# Autodesk Inventor assembly: ASY MSC 080 roсket
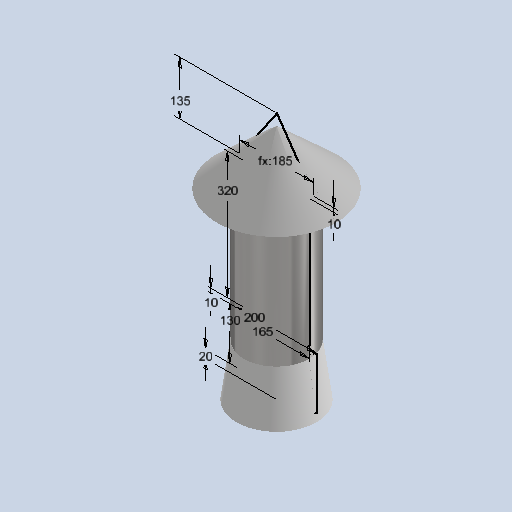
[picture p0: Inventor's stored thumbnail of the model, 512x512]
Saved by Autodesk Inventor 2024.2 (Build 282272000, 272)
## iProperties
Created: 2024-05-19
Part Number: ASY MSC 080 roсket
Document SubType Name: Assembly
Designer: admin
Stock Number: ASY МОО 080 ракета
Author: admin
## Documents named in this file (5)
- C:\Users\pokla\Documents\Inventor\Отстойник осветлитель\Manturovo_Se-clar-Gleb\ASY МОО 060 ракета.iam
- C:\Users\pokla\Documents\Inventor\Отстойник осветлитель\Manturovo_Se-clar-Gleb\МОО DIM 084 ракета эскиз.ipt
- C:\Users\pokla\Documents\Inventor\Отстойник осветлитель\Manturovo_Se-clar-Gleb\ракета\МОО 081 ракета хвост.ipt
- C:\Users\pokla\Documents\Inventor\Отстойник осветлитель\Manturovo_Se-clar-Gleb\ракета\МОО 082 ракета тело.ipt
- C:\Users\pokla\Documents\Inventor\Отстойник осветлитель\Manturovo_Se-clar-Gleb\ракета\МОО 083 ракета нос.ipt
## Components (4 placed, 4 different names)
1. МОО DIM 061  ракета:1
2. МОО 061 ракета хвост:1 — Rigid:1, Mate:2
3. МОО 062 ракета тело:1 — Rigid:1, Rigid:2
4. МОО 063 ракета нос:1 — Rigid:2
## Relationships (3: WeldJoint 2, Mate 1)
- Rigid:1 [WeldJoint]: МОО 061 ракета хвост:1 ↔ МОО 062 ракета тело:1
- Rigid:2 [WeldJoint] (10 mm): МОО 062 ракета тело:1 ↔ МОО 063 ракета нос:1
- Mate:2: МОО 061 ракета хвост:1
